# Autodesk Inventor assembly: tensioner
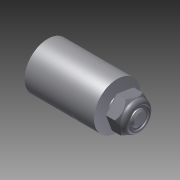
[picture p0: Inventor's stored thumbnail of the model, 180x180]
Saved by Autodesk Inventor 2014 SP1 (Build 180222100, 222)
## iProperties
Created: 2013-08-29
Part Number: tensioner
Document SubType Name: Assembly
Designer: Ryan
Sending System: SolidWorks 2013
Last Author: Ryan
Author: Ryan
## Documents named in this file (5)
- C:\Users\Ryan\Desktop\sw\toss up 1st A bot\inventor drive\tensioner.iam
- C:\Users\Ryan\Desktop\sw\lib\Aperture VEX CAD Library\Hardware\8-32\8-32_1.000.ipt
- C:\Users\Ryan\Desktop\sw\lib\Aperture VEX CAD Library\Spacers\SPACER-0500-0500.ipt
- C:\Users\Ryan\Desktop\sw\lib\Aperture VEX CAD Library\Spacers\spacer-0500-0250.ipt
- C:\Users\Ryan\Desktop\sw\lib\Aperture VEX CAD Library\Hardware\8-32\8-32 Nylock.ipt
## Components (4 placed, 4 different names)
1. 8-32_1-000:1 — Mate:2, Mate:3, Mate:4
2. spacer-0500-0500:1 — Mate:3, Mate:4, Mate:5, Mate:6
3. spacer-0500-0250:1 — Mate:1, Mate:5, Mate:6
4. 8-32 Nylock:1 — Mate:1, Mate:2
## Relationships (6: Mate 6)
- Mate:1 (1.1684 mm): spacer-0500-0250:1 ↔ 8-32 Nylock:1
- Mate:2: 8-32_1-000:1 ↔ 8-32 Nylock:1
- Mate:3: 8-32_1-000:1 ↔ spacer-0500-0500:1
- Mate:4: 8-32_1-000:1 ↔ spacer-0500-0500:1
- Mate:5: spacer-0500-0500:1 ↔ spacer-0500-0250:1
- Mate:6: spacer-0500-0500:1 ↔ spacer-0500-0250:1
## Named parameters: metal = 1.1684 mm
